# Autodesk Inventor assembly: Ensamble
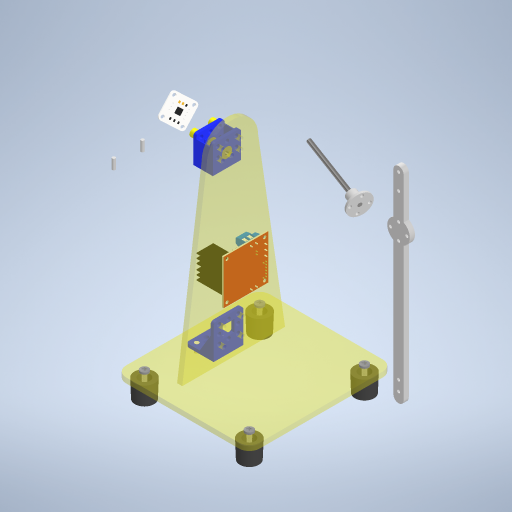
[picture p0: Inventor's stored thumbnail of the model, 512x512]
Saved by Autodesk Inventor 2023.1 (Build 271208000, 208)
## iProperties
Created: 2023-05-03
Part Number: Ensamble
Document SubType Name: Assembly
Designer: felip
Author: felip
## Documents named in this file (16)
- C:\Users\felip\OneDrive\UNAL FORE\SEMESTRE 9\TECNICAS DE CONTROL\PROYECTO\PROYECTO-TDC-INVENTOR\Ensamble.iam
- C:\Users\felip\OneDrive\UNAL FORE\SEMESTRE 9\TECNICAS DE CONTROL\PROYECTO\PROYECTO-TDC-INVENTOR\base.ipt
- C:\Users\felip\OneDrive\UNAL FORE\SEMESTRE 9\TECNICAS DE CONTROL\PROYECTO\PROYECTO-TDC-INVENTOR\SoporteUnion.ipt
- C:\Users\felip\OneDrive\UNAL FORE\SEMESTRE 9\TECNICAS DE CONTROL\PROYECTO\PROYECTO-TDC-INVENTOR\pasador.ipt
- C:\Users\felip\OneDrive\UNAL FORE\SEMESTRE 9\TECNICAS DE CONTROL\PROYECTO\PROYECTO-TDC-INVENTOR\Pata-Goma.ipt
- C:\Users\felip\OneDrive\UNAL FORE\SEMESTRE 9\TECNICAS DE CONTROL\PROYECTO\PROYECTO-TDC-INVENTOR\BaseParal.ipt
- C:\Users\felip\OneDrive\UNAL FORE\SEMESTRE 9\TECNICAS DE CONTROL\PROYECTO\PROYECTO-TDC-INVENTOR\SoporteEncoder.ipt
- C:\Users\felip\OneDrive\UNAL FORE\SEMESTRE 9\TECNICAS DE CONTROL\PROYECTO\PROYECTO-TDC-INVENTOR\L298N_Dual_H_Bruecke.ipt
- C:\Users\felip\OneDrive\UNAL FORE\SEMESTRE 9\TECNICAS DE CONTROL\PROYECTO\PROYECTO-TDC-INVENTOR\M4x14-cheese-head-bolt-phillips-ss.ipt
- C:\Users\felip\OneDrive\UNAL FORE\SEMESTRE 9\TECNICAS DE CONTROL\PROYECTO\PROYECTO-TDC-INVENTOR\rodamiento.ipt
- C:\Users\felip\OneDrive\UNAL FORE\SEMESTRE 9\TECNICAS DE CONTROL\PROYECTO\PROYECTO-TDC-INVENTOR\eje.ipt
- C:\Users\felip\OneDrive\UNAL FORE\SEMESTRE 9\TECNICAS DE CONTROL\PROYECTO\PROYECTO-TDC-INVENTOR\AS5600 v1.ipt
- C:\Users\felip\OneDrive\UNAL FORE\SEMESTRE 9\TECNICAS DE CONTROL\PROYECTO\PROYECTO-TDC-INVENTOR\topito.ipt
- C:\Users\felip\OneDrive\UNAL FORE\SEMESTRE 9\TECNICAS DE CONTROL\PROYECTO\PROYECTO-TDC-INVENTOR\m3.ipt
- C:\Users\felip\OneDrive\UNAL FORE\SEMESTRE 9\TECNICAS DE CONTROL\PROYECTO\PROYECTO-TDC-INVENTOR\brida.ipt
- C:\Users\felip\OneDrive\UNAL FORE\SEMESTRE 9\TECNICAS DE CONTROL\PROYECTO\PROYECTO-TDC-INVENTOR\brazo.ipt
## Components (25 placed, 15 different names)
1. base:1 — Mate:1, Rotational:3, Rotational:4, Rotational:5, Rotational:6, Rotational:7, Rotational:8, Mate:2, Mate:3, Rotational:9, Rotational:10, Rotational:11, Rotational:12
2. SoporteUnion:1 — Mate:1, Rotational:1, Rotational:2, Flush:1, Flush:2, Flush:3, Flush:4
3. pasador:1 — Rotational:1, Rotational:4
4. pasador:2 — Rotational:2, Rotational:3
5. Pata-Goma:1 — Rotational:8
6. Pata-Goma:2 — Rotational:7
7. Pata-Goma:3 — Rotational:5
8. Pata-Goma:4 — Rotational:6
9. BaseParal:1 — Flush:1
10. SoporteEncoder:1 — Flush:2, Mate:2, Flush:4, Insert:1, Insert:2, Insert:3, Insert:4
11. L298N_Dual_H_Bruecke:1 — Mate:3, Flush:3
12. M4x14-cheese-head-bolt-phillips-ss:1 — Rotational:9
13. M4x14-cheese-head-bolt-phillips-ss:2 — Rotational:10
14. M4x14-cheese-head-bolt-phillips-ss:3 — Rotational:12
15. M4x14-cheese-head-bolt-phillips-ss:5 — Rotational:11
16. rodamiento:1 — Insert:2
17. rodamiento:2 — Insert:1
18. eje:1 — Insert:5
19. AS5600 v1:1
20. topito:1 — Insert:3
21. topito:2 — Insert:4
22. m3:1
23. m3:2
24. brida:1 — Insert:5
25. brazo:1
## Relationships (24: RevoluteJoint 12, Insert 5, Flush 4, Mate 3)
- Mate:1: base:1 ↔ SoporteUnion:1
- Rotational:1 [RevoluteJoint]: SoporteUnion:1 ↔ pasador:1
- Rotational:2 [RevoluteJoint]: SoporteUnion:1 ↔ pasador:2
- Rotational:3 [RevoluteJoint]: base:1 ↔ pasador:2
- Rotational:4 [RevoluteJoint]: base:1 ↔ pasador:1
- Rotational:5 [RevoluteJoint]: base:1 ↔ Pata-Goma:3
- Rotational:6 [RevoluteJoint]: base:1 ↔ Pata-Goma:4
- Rotational:7 [RevoluteJoint]: base:1 ↔ Pata-Goma:2
- Rotational:8 [RevoluteJoint]: base:1 ↔ Pata-Goma:1
- Flush:1: SoporteUnion:1 ↔ BaseParal:1
- Flush:2: SoporteUnion:1 ↔ SoporteEncoder:1
- Mate:2 (157 mm): base:1 ↔ SoporteEncoder:1
- Mate:3 (38 mm): base:1 ↔ L298N_Dual_H_Bruecke:1
- Flush:3 (2.5 mm): SoporteUnion:1 ↔ L298N_Dual_H_Bruecke:1
- Rotational:9 [RevoluteJoint]: base:1 ↔ M4x14-cheese-head-bolt-phillips-ss:1
- Rotational:10 [RevoluteJoint]: base:1 ↔ M4x14-cheese-head-bolt-phillips-ss:2
- Rotational:11 [RevoluteJoint]: base:1 ↔ M4x14-cheese-head-bolt-phillips-ss:5
- Rotational:12 [RevoluteJoint]: base:1 ↔ M4x14-cheese-head-bolt-phillips-ss:3
- Flush:4 (0.75 mm): SoporteUnion:1 ↔ SoporteEncoder:1
- Insert:1: SoporteEncoder:1 ↔ rodamiento:2
- Insert:2: SoporteEncoder:1 ↔ rodamiento:1
- Insert:3: SoporteEncoder:1 ↔ topito:1
- Insert:4: SoporteEncoder:1 ↔ topito:2
- Insert:5: eje:1 ↔ brida:1
